# Autodesk Inventor assembly: КВ33.044.200 - Каретка оси Х
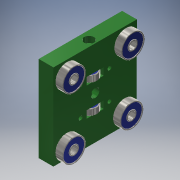
[picture p0: Inventor's stored thumbnail of the model, 180x180]
Saved by Autodesk Inventor 2019 (Build 230136000, 136)
## iProperties
Created: 2019-07-16
Part Number: КВ33.044.200 - Каретка оси Х
Material: Типовые
Document SubType Name: Assembly
Designer: Петров Иван
Author: Петров Иван
## Documents named in this file (4)
- C:\Users\user\Documents\Kvantoriada2019\optimal_gripper\hardware\КВ33.044.200 - Каретка оси Х.iam
- C:\Users\user\Documents\Kvantoriada2019\optimal_gripper\hardware\КВ33.044.201 - Щека каретки.ipt
- C:\Users\user\Documents\Kvantoriada2019\optimal_gripper\hardware\Стандартные изделия\Подшипник 626Z.ipt
- C:\Users\user\Documents\Kvantoriada2019\optimal_gripper\hardware\Стандартные изделия\Подшипник 624Z.ipt
## Components (7 placed, 3 different names)
1. КВ33.044.201 - Щека каретки:1 — Совмещение:1, Совмещение:2, Совмещение:3, Совмещение:4, Совмещение:5, Совмещение:6, Совмещение:7, Совмещение:8, Совмещение:9, Совмещение:10, Совмещение:11, Совмещение:12
2. Подшипник 626Z:1 — Совмещение:1, Совмещение:2
3. Подшипник 626Z:2 — Совмещение:3, Совмещение:6
4. Подшипник 626Z:3 — Совмещение:5, Совмещение:8
5. Подшипник 626Z:4 — Совмещение:4, Совмещение:7
6. Подшипник 624Z:1 — Совмещение:9, Совмещение:10
7. Подшипник 624Z:2 — Совмещение:11, Совмещение:12
## Relationships (12: Mate 12)
- Совмещение:1 [Mate]: КВ33.044.201 - Щека каретки:1 ↔ Подшипник 626Z:1
- Совмещение:2 [Mate] (1 mm): КВ33.044.201 - Щека каретки:1 ↔ Подшипник 626Z:1
- Совмещение:3 [Mate]: КВ33.044.201 - Щека каретки:1 ↔ Подшипник 626Z:2
- Совмещение:4 [Mate]: КВ33.044.201 - Щека каретки:1 ↔ Подшипник 626Z:4
- Совмещение:5 [Mate]: КВ33.044.201 - Щека каретки:1 ↔ Подшипник 626Z:3
- Совмещение:6 [Mate] (1 mm): КВ33.044.201 - Щека каретки:1 ↔ Подшипник 626Z:2
- Совмещение:7 [Mate] (1 mm): КВ33.044.201 - Щека каретки:1 ↔ Подшипник 626Z:4
- Совмещение:8 [Mate]: КВ33.044.201 - Щека каретки:1 ↔ Подшипник 626Z:3
- Совмещение:9 [Mate]: КВ33.044.201 - Щека каретки:1 ↔ Подшипник 624Z:1
- Совмещение:10 [Mate] (0.5 mm): КВ33.044.201 - Щека каретки:1 ↔ Подшипник 624Z:1
- Совмещение:11 [Mate]: КВ33.044.201 - Щека каретки:1 ↔ Подшипник 624Z:2
- Совмещение:12 [Mate] (0.5 mm): КВ33.044.201 - Щека каретки:1 ↔ Подшипник 624Z:2
